# Autodesk Inventor assembly: BC-100004
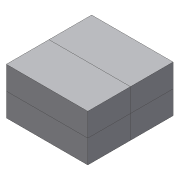
[picture p0: Inventor's stored thumbnail of the model, 180x180]
Saved by Autodesk Inventor 2016 (Build 200138000, 138)
## iProperties
Created: 2015-10-05
Part Number: BC-100004
Document SubType Name: Assembly
Designer: Insira seu nome aqui!
Author: Insira seu nome aqui!
## Documents named in this file (2)
- D:\ARQ\Basilio\LNLS-2\Anel\Dipolos\BC-3T\Dipolo 3T e 1T\Prototipo 1\Projeto Mecanico\BC-100004.iam
- D:\ARQ\Basilio\LNLS-2\Anel\Dipolos\BC-3T\Dipolo 3T e 1T\Prototipo 1\Projeto Mecanico\NdFeB.ipt
## Components (4 placed, 1 different names)
1. NdFeB:1 — Mate:1, Flush:1, Flush:2, Mate:2, Flush:6, Flush:7, Flush:8
2. NdFeB:2 — Mate:2, Flush:3, Mate:4
3. NdFeB:3 — Mate:3, Flush:3, Mate:4, Flush:4, Flush:5
4. NdFeB:4 — Mate:1, Flush:1, Flush:2, Mate:3, Flush:4, Flush:5
## Relationships (12: Flush 8, Mate 4)
- Mate:1: NdFeB:1 ↔ NdFeB:4
- Flush:1: NdFeB:1 ↔ NdFeB:4
- Flush:2: NdFeB:1 ↔ NdFeB:4
- Mate:2: NdFeB:1 ↔ NdFeB:2
- Mate:3: NdFeB:3 ↔ NdFeB:4
- Flush:3: NdFeB:2 ↔ NdFeB:3
- Mate:4: NdFeB:2 ↔ NdFeB:3
- Flush:4: NdFeB:3 ↔ NdFeB:4
- Flush:5: NdFeB:3 ↔ NdFeB:4
- Flush:6: NdFeB:1
- Flush:7 (27.5 mm): NdFeB:1
- Flush:8: NdFeB:1
